# Autodesk Inventor assembly: Crossbow CNC VC4_T1_V2_assy
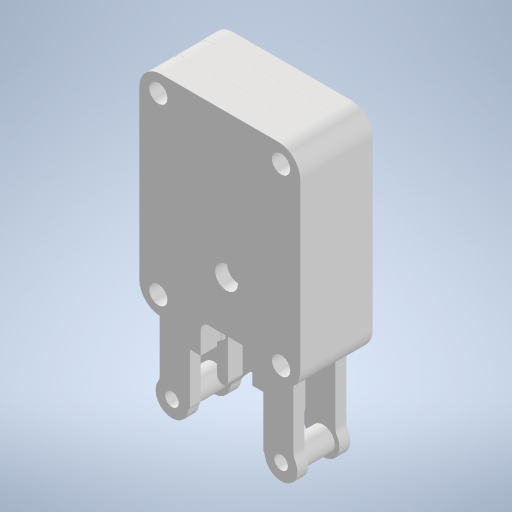
[picture p0: Inventor's stored thumbnail of the model, 512x512]
Saved by Autodesk Inventor 2024 (Build 280153000, 153)
## iProperties
Created: 2026-03-14
Part Number: Crossbow CNC VC4_T1_V2_assy
Document SubType Name: Assembly
Designer: RidDleZ
Author: RidDleZ
## Documents named in this file (5)
- C:\Users\RidDleZ\Desktop\Reprap\RatRig\IDEX\RidDleZEazyIDEX\34Hybrid\VC4Toolhead\crossbow_cutter_VC4\Crossbow CNC VC4_LGX_LITE_UNI_assy.iam
- C:\Users\RidDleZ\Desktop\Reprap\RatRig\IDEX\RidDleZEazyIDEX\34Hybrid\VC4Toolhead\crossbow_cutter_VC4\Crossbow CNC VC4_LGX_LITE_UNI_spacer_v2.ipt
- C:\Users\RidDleZ\Desktop\Reprap\RatRig\IDEX\RidDleZEazyIDEX\34Hybrid\VC4Toolhead\crossbow_cutter_VC4\Crossbow CNC VC4_LGX_LITE_UNI_body_v2.ipt
- Crossbow CNC VC4_T1_body_v2.ipt
- C:\Users\RidDleZ\Desktop\Reprap\RatRig\IDEX\RidDleZEazyIDEX\34Hybrid\VC4Toolhead\crossbow_cutter_VC4\Crossbow CNC VC4_LGX_LITE_UNI_holder_V2.ipt
## Components (3 placed, 3 different names)
1. Crossbow CNC VC4_LGX_LITE_UNI_spacer_v2:1 — Mate:1
2. Crossbow CNC VC4_LGX_LITE_UNI_body_v2:1 — Mate:1, Mate:2
3. Crossbow CNC VC4_LGX_LITE_UNI_holder_V2:1 — Mate:2
## Relationships (2: Mate 2)
- Mate:1: Crossbow CNC VC4_LGX_LITE_UNI_spacer_v2:1 ↔ Crossbow CNC VC4_LGX_LITE_UNI_body_v2:1
- Mate:2: Crossbow CNC VC4_LGX_LITE_UNI_body_v2:1 ↔ Crossbow CNC VC4_LGX_LITE_UNI_holder_V2:1
